# Autodesk Inventor assembly: HH-3465 Assembly
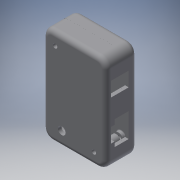
[picture p0: Inventor's stored thumbnail of the model, 180x180]
Saved by Autodesk Inventor 2018.3 (Build 223284000, 284)
## iProperties
Created: 2018-10-27
Part Number: HH-3465 Assembly
Document SubType Name: Assembly
Designer: birtj
Author: birtj
## Documents named in this file (3)
- C:\Users\birtj\OneDrive\C64 Cassette Adapter\Data\Enclosures\HH-3465 Inspired Model\HH-3465 Assembly.iam
- C:\Users\birtj\OneDrive\C64 Cassette Adapter\Data\Enclosures\HH-3465 Inspired Model\Bottom.ipt
- C:\Users\birtj\OneDrive\C64 Cassette Adapter\Data\Enclosures\HH-3465 Inspired Model\Top.ipt
## Components (2 placed, 2 different names)
1. Bottom:1 — Mate:1, Flush:1, Flush:2
2. Top:1 — Mate:1, Flush:1, Flush:2
## Relationships (3: Flush 2, Mate 1)
- Mate:1: Bottom:1 ↔ Top:1
- Flush:1: Bottom:1 ↔ Top:1
- Flush:2: Bottom:1 ↔ Top:1
